# Autodesk Inventor assembly: 4t2000
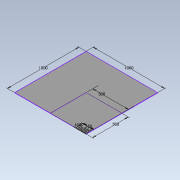
[picture p0: Inventor's stored thumbnail of the model, 180x180]
Saved by Autodesk Inventor 2020.3 (Build 243373000, 373)
## iProperties
Created: 2020-05-22
Part Number: 4t2000
Document SubType Name: Assembly
Designer: aoyama
Author: aoyama
## Documents named in this file (6)
- C:\Users\aoyam\Desktop\SRDC_local\Inventor\二年機\Geminiβ\4t2000.iam
- C:\Users\aoyam\Desktop\SRDC_local\Inventor\二年機\AL板サイズ測定板.ipt
- C:\Users\aoyam\Desktop\SRDC_local\Inventor\二年機\Geminiβ\汎用部品\ｍ2歯数9ギアd3.99.ipt
- C:\Users\aoyam\Desktop\SRDC_local\Inventor\二年機\Geminiβ\汎用部品\ｍ2歯数25ギアネジ.ipt
- C:\Users\aoyam\Desktop\SRDC_local\Inventor\二年機\Geminiβ\脚\中間ユニット\中間ギア抑え.ipt
- C:\Users\aoyam\Desktop\SRDC_local\Inventor\二年機\Geminiβ\脚\中間ユニット\脚中間フレームカム3.ipt
## Components (9 placed, 5 different names)
1. AL板サイズ測定板:1 — メイト:1, メイト:2, メイト:3, メイト:4, メイト:6, メイト:7, メイト:8, メイト:9
2. ｍ2歯数9ギアd3.99:1 — メイト:1
3. ｍ2歯数9ギアd3.99:2 — メイト:2
4. ｍ2歯数25ギアネジ:1 — メイト:4
5. ｍ2歯数25ギアネジ:2 — メイト:3
6. 中間ギア抑え:1 — メイト:7
7. 中間ギア抑え:2 — メイト:6
8. 脚中間フレームカム3:1 — メイト:8
9. 脚中間フレームカム3:2 — メイト:9
## Relationships (8: Mate 8)
- メイト:1 [Mate]: AL板サイズ測定板:1 ↔ ｍ2歯数9ギアd3.99:1
- メイト:2 [Mate]: AL板サイズ測定板:1 ↔ ｍ2歯数9ギアd3.99:2
- メイト:3 [Mate]: AL板サイズ測定板:1 ↔ ｍ2歯数25ギアネジ:2
- メイト:4 [Mate]: AL板サイズ測定板:1 ↔ ｍ2歯数25ギアネジ:1
- メイト:6 [Mate]: AL板サイズ測定板:1 ↔ 中間ギア抑え:2
- メイト:7 [Mate]: AL板サイズ測定板:1 ↔ 中間ギア抑え:1
- メイト:8 [Mate]: AL板サイズ測定板:1 ↔ 脚中間フレームカム3:1
- メイト:9 [Mate]: AL板サイズ測定板:1 ↔ 脚中間フレームカム3:2
